# Autodesk Inventor assembly: 千斤頂
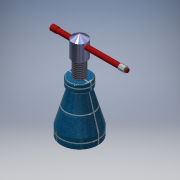
[picture p0: Inventor's stored thumbnail of the model, 180x180]
Saved by Autodesk Inventor 2017 (Build 210142000, 142)
## iProperties
Part Number: 千斤頂
Material: 一般
Document SubType Name: Assembly
Designer: user
Author: user
## Documents named in this file (6)
- C:\Users\user\Desktop\千斤頂.iam
- C:\Users\user\Desktop\A.ipt
- C:\Users\user\Desktop\A2.ipt
- C:\Users\user\Desktop\B.ipt
- C:\Users\user\Desktop\C.ipt
- C:\Users\user\Desktop\零件7.ipt
## Components (5 placed, 5 different names)
1. C:1 — 剛性:1
2. B:1 — 剛性:1, 圓柱:1, 貼合:1
3. A:1 — 圓柱:1, 旋轉:1, 貼合:1
4. A2:1 — 旋轉:1
5. 零件7:1
## Relationships (4: WeldJoint 1, CylindricalJoint 1, RevoluteJoint 1, Mate 1)
- 剛性:1 [WeldJoint] (4 mm): C:1 ↔ B:1
- 圓柱:1 [CylindricalJoint]: B:1 ↔ A:1
- 旋轉:1 [RevoluteJoint] (-2 mm): A:1 ↔ A2:1
- 貼合:1 [Mate]: B:1 ↔ A:1
